# Autodesk Inventor assembly: Base_Roulante_Ammovible
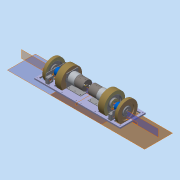
[picture p0: Inventor's stored thumbnail of the model, 180x180]
Saved by Autodesk Inventor 2016 (Build 200138000, 138)
## iProperties
Created: 2012-09-17
Part Number: Base_Roulante_Ammovible
Document SubType Name: Assembly
Designer: Aegir
Author: Aegir
## Documents named in this file (22)
- C:\Users\Aegir\Documents\robotik 2017\git\base roulante_v2\conception\Base_Roulante_Ammovible.iam
- C:\Users\Aegir\Documents\robotik 2017\git\base roulante_v2\conception\Base_Moteur.ipt
- C:\Users\Aegir\Documents\robotik 2017\git\base roulante_v2\conception\Ammortisseurv2.iam
- C:\Users\Aegir\Documents\robotik 2017\git\base roulante_v2\conception\ensemble_moteur.iam
- C:\Users\Aegir\Documents\robotik 2017\git\base roulante_v2\conception\moyeux_expansible.ipt
- C:\Users\Aegir\Documents\robotik 2017\git\base roulante_v2\conception\Colson_Wheel_3in_x_7_8in.ipt
- C:\Users\Aegir\Documents\robotik 2017\git\base roulante_v2\conception\palier_roulement_bras.ipt
- C:\Users\Aegir\Documents\Inventor\Content Center Files\R2016\fr-FR\ISO 2795  C\ISO 2795 - 5 x 9 x 8C.ipt
- C:\Users\Aegir\Documents\robotik 2017\git\base roulante_v2\conception\crochet.ipt
- C:\Users\Aegir\Documents\robotik 2017\git\base roulante_v2\conception\T40_hub_40mm_1screw.ipt
- C:\Users\Aegir\Documents\robotik 2017\git\base roulante_v2\conception\T40_Wheel_2_875in_x_0_5in.ipt
- C:\Users\Aegir\Documents\robotik 2017\git\base roulante_v2\conception\Base_Moteur_MIR.ipt
- C:\Users\Aegir\Documents\robotik 2017\git\base roulante_v2\conception\ensemble_moteur_MIR.iam
- C:\Users\Aegir\Documents\robotik 2017\git\base roulante_v2\conception\moyeux_expansible_MIR.ipt
- C:\Users\Aegir\Documents\robotik 2017\git\base roulante_v2\conception\Colson_Wheel_3in_x_7_8in_MIR.ipt
- C:\Users\Aegir\Documents\robotik 2017\git\base roulante_v2\conception\crochet_MIR.ipt
- C:\Users\Aegir\Documents\robotik 2017\git\base roulante_v2\conception\palier_roulement_bras_MIR1.ipt
- C:\Users\Aegir\Documents\robotik 2017\git\base roulante_v2\conception\bras_final_codeur.ipt
- C:\Users\Aegir\Documents\robotik 2017\git\base roulante_v2\conception\Ammortisseurv2_MIR1.iam
- C:\Users\Aegir\Documents\robotik 2017\git\base roulante_v2\conception\T40_hub_40mm_1screw_MIR1.ipt
- C:\Users\Aegir\Documents\robotik 2017\git\base roulante_v2\conception\T40_Wheel_2_875in_x_0_5in_MIR1.ipt
- C:\Users\Aegir\Documents\robotik 2017\git\base roulante_v2\conception\bras_final_codeur_MIR.ipt
## Components (22 placed, 21 different names)
1. Base_Moteur.1 — Placage:4, Affleurement:3, Placage:18, Affleurement:13, Angle:2, Affleurement:16, Placage:33, Affleurement:17
2. Ammortisseurv2.1 [sub-assembly] — Placage:30, Placage:31, Placage:32, Placage:53
3. ensemble_moteur:2 [sub-assembly] — Placage:4, Affleurement:3, Placage:8, Affleurement:4
4. moyeux_expansible:2 — Placage:8, Affleurement:4, Placage:9, Affleurement:7
5. Colson_Wheel_3in_x_7_8in:1 — Placage:9, Affleurement:7, Placage:19
6. ISO 2795 (Cylindriques) 5 x 9 x 8:1 — Placage:34, Affleurement:18, Placage:52
7. crochet:2 — Placage:18, Affleurement:13
8. T40_hub_40mm_1screw:1 — Placage:28, Placage:29, Placage:31, Placage:32, Placage:36
9. T40_Wheel_2_875in_x_0_5in:1 — Placage:28, Placage:29, Tangente:1, Placage:36
10. palier_roulement_bras:1 — Placage:33, Affleurement:17, Placage:34, Affleurement:18, Placage:51
11. Base_Moteur_MIR:1 — Affleurement:21, Placage:37, Affleurement:24, Placage:40, Angle:3, Affleurement:25
12. ensemble_moteur_MIR:1 [sub-assembly] — Affleurement:21, Placage:37, Affleurement:22, Placage:38
13. moyeux_expansible_MIR:1 — Affleurement:22, Placage:38, Affleurement:23, Placage:39
14. Colson_Wheel_3in_x_7_8in_MIR:1 — Affleurement:23, Placage:39, Placage:41
15. crochet_MIR:1 — Affleurement:24, Placage:40
16. ISO 2795 (Cylindriques) 5 x 9 x 8:2 — Affleurement:26, Placage:49
17. palier_roulement_bras_MIR1:1 — Affleurement:26, Placage:49
18. bras_final_codeur:1 — Placage:51, Placage:52, Placage:53
19. Ammortisseurv2_MIR1:1 [sub-assembly] — Placage:54, Placage:55, Placage:56, Placage:60
20. T40_hub_40mm_1screw_MIR1:1 — Placage:55, Placage:56, Placage:57, Placage:58, Placage:59
21. T40_Wheel_2_875in_x_0_5in_MIR1:1 — Placage:57, Placage:58, Placage:59, Tangente:2
22. bras_final_codeur_MIR:1 — Placage:60
## Relationships (48: Mate 31, Flush 13, Angle 2, Tangent 2)
- Placage:4 [Mate]: Base_Moteur.1 ↔ ensemble_moteur:2
- Affleurement:3 [Flush]: Base_Moteur.1 ↔ ensemble_moteur:2
- Placage:8 [Mate]: ensemble_moteur:2 ↔ moyeux_expansible:2
- Affleurement:4 [Flush]: ensemble_moteur:2 ↔ moyeux_expansible:2
- Placage:9 [Mate]: moyeux_expansible:2 ↔ Colson_Wheel_3in_x_7_8in:1
- Affleurement:7 [Flush] (4 mm): moyeux_expansible:2 ↔ Colson_Wheel_3in_x_7_8in:1
- Placage:18 [Mate]: Base_Moteur.1 ↔ crochet:2
- Affleurement:13 [Flush] (5 mm): Base_Moteur.1 ↔ crochet:2
- Placage:19 [Mate]: Colson_Wheel_3in_x_7_8in:1
- Placage:20 [Mate]
- Angle:2 (180 deg): Base_Moteur.1
- Placage:28 [Mate]: T40_hub_40mm_1screw:1 ↔ T40_Wheel_2_875in_x_0_5in:1
- Placage:29 [Mate]: T40_hub_40mm_1screw:1 ↔ T40_Wheel_2_875in_x_0_5in:1
- Affleurement:16 [Flush] (15 mm): Base_Moteur.1
- Tangente:1: T40_Wheel_2_875in_x_0_5in:1
- Placage:30 [Mate]: Ammortisseurv2.1
- Placage:31 [Mate]: Ammortisseurv2.1 ↔ T40_hub_40mm_1screw:1
- Placage:32 [Mate] (6 mm): Ammortisseurv2.1 ↔ T40_hub_40mm_1screw:1
- Placage:33 [Mate]: Base_Moteur.1 ↔ palier_roulement_bras:1
- Affleurement:17 [Flush] (3 mm): Base_Moteur.1 ↔ palier_roulement_bras:1
- Placage:34 [Mate]: ISO 2795 (Cylindriques) 5 x 9 x 8:1 ↔ palier_roulement_bras:1
- Affleurement:18 [Flush]: ISO 2795 (Cylindriques) 5 x 9 x 8:1 ↔ palier_roulement_bras:1
- Placage:36 [Mate]: T40_hub_40mm_1screw:1 ↔ T40_Wheel_2_875in_x_0_5in:1
- Affleurement:21 [Flush]: Base_Moteur_MIR:1 ↔ ensemble_moteur_MIR:1
- Placage:37 [Mate]: Base_Moteur_MIR:1 ↔ ensemble_moteur_MIR:1
- Affleurement:22 [Flush]: ensemble_moteur_MIR:1 ↔ moyeux_expansible_MIR:1
- Placage:38 [Mate]: ensemble_moteur_MIR:1 ↔ moyeux_expansible_MIR:1
- Affleurement:23 [Flush] (4 mm): moyeux_expansible_MIR:1 ↔ Colson_Wheel_3in_x_7_8in_MIR:1
- Placage:39 [Mate]: moyeux_expansible_MIR:1 ↔ Colson_Wheel_3in_x_7_8in_MIR:1
- Affleurement:24 [Flush] (5 mm): Base_Moteur_MIR:1 ↔ crochet_MIR:1
- Placage:40 [Mate]: Base_Moteur_MIR:1 ↔ crochet_MIR:1
- Placage:41 [Mate]: Colson_Wheel_3in_x_7_8in_MIR:1
- Placage:43 [Mate]
- Angle:3 (-180 deg): Base_Moteur_MIR:1
- Affleurement:25 [Flush] (15 mm): Base_Moteur_MIR:1
- Affleurement:26 [Flush]: ISO 2795 (Cylindriques) 5 x 9 x 8:2 ↔ palier_roulement_bras_MIR1:1
- Placage:49 [Mate]: ISO 2795 (Cylindriques) 5 x 9 x 8:2 ↔ palier_roulement_bras_MIR1:1
- Placage:51 [Mate]: palier_roulement_bras:1 ↔ bras_final_codeur:1
- Placage:52 [Mate]: ISO 2795 (Cylindriques) 5 x 9 x 8:1 ↔ bras_final_codeur:1
- Placage:53 [Mate]: Ammortisseurv2.1 ↔ bras_final_codeur:1
- Placage:54 [Mate]: Ammortisseurv2_MIR1:1
- Placage:55 [Mate] (6 mm): Ammortisseurv2_MIR1:1 ↔ T40_hub_40mm_1screw_MIR1:1
- Placage:56 [Mate]: Ammortisseurv2_MIR1:1 ↔ T40_hub_40mm_1screw_MIR1:1
- Placage:57 [Mate]: T40_hub_40mm_1screw_MIR1:1 ↔ T40_Wheel_2_875in_x_0_5in_MIR1:1
- Placage:58 [Mate]: T40_hub_40mm_1screw_MIR1:1 ↔ T40_Wheel_2_875in_x_0_5in_MIR1:1
- Placage:59 [Mate]: T40_hub_40mm_1screw_MIR1:1 ↔ T40_Wheel_2_875in_x_0_5in_MIR1:1
- Tangente:2: T40_Wheel_2_875in_x_0_5in_MIR1:1
- Placage:60 [Mate]: Ammortisseurv2_MIR1:1 ↔ bras_final_codeur_MIR:1
